# Autodesk Inventor assembly: FrameV2
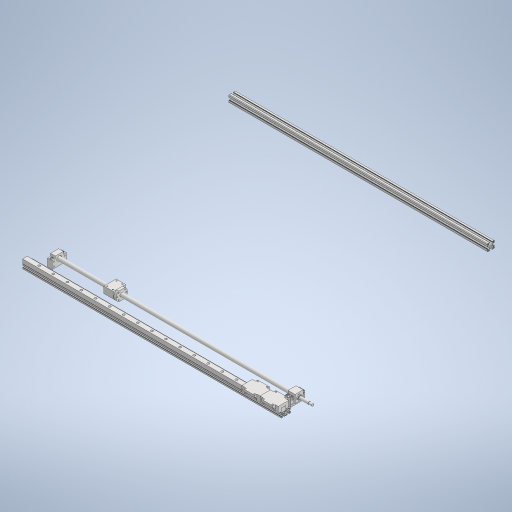
[picture p0: Inventor's stored thumbnail of the model, 512x512]
Saved by Autodesk Inventor 2023 (Build 270158000, 158)
## iProperties
Created: 2022-05-01
Part Number: FrameV2
Document SubType Name: Assembly
Designer: plebbb
Author: plebbb
## Documents named in this file (10)
- D:\Users\plebbb\Desktop\CNC_Project\FrameV2.iam
- D:\Users\plebbb\Desktop\CNC_Project\HGW20CC_Rail_800mm.ipt
- D:\Users\plebbb\Desktop\CNC_Project\HGW20CC_Slider.ipt
- D:\Users\plebbb\Desktop\CNC_Project\SFU1605_800mm.ipt
- D:\Users\plebbb\Desktop\CNC_Project\SFU1605_Nut.ipt
- D:\Users\plebbb\Desktop\CNC_Project\DSG16H.ipt
- D:\Users\plebbb\Desktop\CNC_Project\3030_Extrusion.ipt
- D:\Users\plebbb\Desktop\CNC_Project\BF12.ipt
- D:\Users\plebbb\Desktop\CNC_Project\BK12.ipt
- D:\Users\plebbb\Desktop\CNC_Project\2040_Extrusion.ipt
## Components (10 placed, 9 different names)
1. HGW20CC_Rail_800mm:1 — Mate:1, Mate:2, Mate:3, Mate:4, Flush:1, Flush:22, Mate:24, Flush:23
2. HGW20CC_Slider:1 — Mate:1, Mate:2, Mate:5
3. SFU1605_800mm:1 — Mate:9, Mate:16, Flush:19, Mate:17, Mate:18
4. SFU1605_Nut:1 — Mate:6, Mate:7, Mate:8, Mate:9
5. HGW20CC_Slider:2 — Mate:3, Mate:4, Mate:5, Flush:1
6. DSG16H:1 — Mate:6, Mate:7, Mate:8, Mate:20, Angle:1
7. 3030_Extrusion:7
8. BF12:1 — Mate:17, Mate:18, Mate:20
9. BK12:1 — Mate:16, Flush:19, Angle:1
10. 2040_Extrusion:1 — Flush:22, Mate:24, Flush:23
## Relationships (19: Mate 14, Flush 4, Angle 1)
- Mate:1: HGW20CC_Rail_800mm:1 ↔ HGW20CC_Slider:1
- Mate:2: HGW20CC_Rail_800mm:1 ↔ HGW20CC_Slider:1
- Mate:3: HGW20CC_Rail_800mm:1 ↔ HGW20CC_Slider:2
- Mate:4: HGW20CC_Rail_800mm:1 ↔ HGW20CC_Slider:2
- Mate:5: HGW20CC_Slider:1 ↔ HGW20CC_Slider:2
- Mate:6: SFU1605_Nut:1 ↔ DSG16H:1
- Mate:7: SFU1605_Nut:1 ↔ DSG16H:1
- Mate:8: SFU1605_Nut:1 ↔ DSG16H:1
- Mate:9: SFU1605_800mm:1 ↔ SFU1605_Nut:1
- Flush:1: HGW20CC_Rail_800mm:1 ↔ HGW20CC_Slider:2
- Mate:16: SFU1605_800mm:1 ↔ BK12:1
- Flush:19: SFU1605_800mm:1 ↔ BK12:1
- Mate:17: SFU1605_800mm:1 ↔ BF12:1
- Mate:18: SFU1605_800mm:1 ↔ BF12:1
- Mate:20: DSG16H:1 ↔ BF12:1
- Angle:1 (0 deg): DSG16H:1 ↔ BK12:1
- Flush:22: HGW20CC_Rail_800mm:1 ↔ 2040_Extrusion:1
- Mate:24: HGW20CC_Rail_800mm:1 ↔ 2040_Extrusion:1
- Flush:23: HGW20CC_Rail_800mm:1 ↔ 2040_Extrusion:1
